# Autodesk Inventor assembly: płyta_bazowa_elewacji
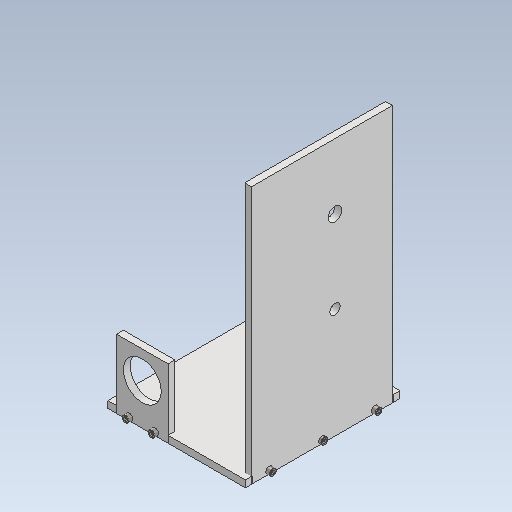
[picture p0: Inventor's stored thumbnail of the model, 512x512]
Saved by Autodesk Inventor 2020 (Build 240168000, 168)
## iProperties
Created: 2020-08-17
Part Number: płyta_bazowa_elewacji
Document SubType Name: Assembly
Designer: Hesekiel
Author: Hesekiel
## Documents named in this file (11)
- C:\Users\Hesekiel\Desktop\Equatorial-Mount-MUM\Mechanika\Mechanizm elewacji Filip\CAD\płyta_bazowa_elewacji.iam
- C:\Users\Hesekiel\Desktop\Equatorial-Mount-MUM\Mechanika\Mechanizm elewacji Filip\CAD\baza.ipt
- C:\Users\Hesekiel\Desktop\Equatorial-Mount-MUM\Mechanika\Mechanizm elewacji Filip\CAD\blok_łożyska.ipt
- C:\Users\Hesekiel\Desktop\Equatorial-Mount-MUM\Mechanika\Mechanizm elewacji Filip\CAD\płyta_bazowa_elewacji\Design Accelerator\Bolted Connection3.iam
- C:\Users\Hesekiel\Desktop\Equatorial-Mount-MUM\Mechanika\Mechanizm elewacji Filip\CAD\płyta_bazowa_elewacji\Design Accelerator\Bolted Connection4.iam
- C:\Users\Hesekiel\Desktop\Equatorial-Mount-MUM\Mechanika\Mechanizm elewacji Filip\CAD\płyta_bazowa_elewacji\Design Accelerator\Bolted Connection5.iam
- C:\Users\Hesekiel\Desktop\Equatorial-Mount-MUM\Mechanika\Mechanizm elewacji Filip\CAD\płyta_bazowa_elewacji\Design Accelerator\Bolted Connection6.iam
- C:\Users\Hesekiel\Desktop\Equatorial-Mount-MUM\Mechanika\Mechanizm elewacji Filip\CAD\płyta_boczna_obudowy.ipt
- C:\Users\Hesekiel\Desktop\Equatorial-Mount-MUM\Mechanika\Mechanizm elewacji Filip\CAD\płyta_bazowa_elewacji\Design Accelerator\Bolted Connection7.iam
- C:\Users\Hesekiel\Desktop\Equatorial-Mount-MUM\Mechanika\Mechanizm elewacji Filip\CAD\płyta_bazowa_elewacji\Design Accelerator\Bolted Connection8.iam
- C:\Users\Hesekiel\Desktop\Equatorial-Mount-MUM\Mechanika\Mechanizm elewacji Filip\CAD\płyta_bazowa_elewacji\Design Accelerator\Bolted Connection9.iam
## Components (11 placed, 4 different names)
1. baza:1 — Mate:1, Mate:2, Mate:3, Mate:4, Mate:5, Mate:6, Flush:1, Mate:15, Mate:16
2. blok_łożyska:1 — Mate:4, Mate:5, Mate:6, Mate:11, Mate:12, Mate:13, Mate:14
3. blok_łożyska:2 — Mate:1, Mate:2, Mate:3, Mate:7, Mate:8, Mate:9, Mate:10
4. Bolted Connection:1 [sub-assembly] — Mate:7, Mate:8
5. Bolted Connection:2 [sub-assembly] — Mate:9, Mate:10
6. Bolted Connection:3 [sub-assembly] — Mate:11, Mate:12
7. Bolted Connection:4 [sub-assembly] — Mate:13, Mate:14
8. płyta_boczna_obudowy:1 — Flush:1, Mate:15, Mate:16, Mate:17, Mate:18, Mate:19, Mate:20, Mate:21, Mate:22
9. Bolted Connection:5 [sub-assembly] — Mate:17, Mate:18
10. Bolted Connection:6 [sub-assembly] — Mate:19, Mate:20
11. Bolted Connection:7 [sub-assembly] — Mate:21, Mate:22
## Relationships (23: Mate 22, Flush 1)
- Mate:1: baza:1 ↔ blok_łożyska:2
- Mate:2: baza:1 ↔ blok_łożyska:2
- Mate:3: baza:1 ↔ blok_łożyska:2
- Mate:4: baza:1 ↔ blok_łożyska:1
- Mate:5: baza:1 ↔ blok_łożyska:1
- Mate:6: baza:1 ↔ blok_łożyska:1
- Mate:7: blok_łożyska:2 ↔ Bolted Connection:1
- Mate:8: blok_łożyska:2 ↔ Bolted Connection:1
- Mate:9: blok_łożyska:2 ↔ Bolted Connection:2
- Mate:10: blok_łożyska:2 ↔ Bolted Connection:2
- Mate:11: blok_łożyska:1 ↔ Bolted Connection:3
- Mate:12: blok_łożyska:1 ↔ Bolted Connection:3
- Mate:13: blok_łożyska:1 ↔ Bolted Connection:4
- Mate:14: blok_łożyska:1 ↔ Bolted Connection:4
- Flush:1: baza:1 ↔ płyta_boczna_obudowy:1
- Mate:15: baza:1 ↔ płyta_boczna_obudowy:1
- Mate:16: baza:1 ↔ płyta_boczna_obudowy:1
- Mate:17: płyta_boczna_obudowy:1 ↔ Bolted Connection:5
- Mate:18: płyta_boczna_obudowy:1 ↔ Bolted Connection:5
- Mate:19: płyta_boczna_obudowy:1 ↔ Bolted Connection:6
- Mate:20: płyta_boczna_obudowy:1 ↔ Bolted Connection:6
- Mate:21: płyta_boczna_obudowy:1 ↔ Bolted Connection:7
- Mate:22: płyta_boczna_obudowy:1 ↔ Bolted Connection:7
